# Autodesk Inventor assembly: hubRings
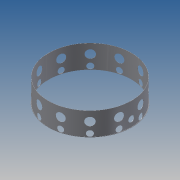
[picture p0: Inventor's stored thumbnail of the model, 180x180]
Saved by Autodesk Inventor 2014 SP1 (Build 180222100, 222)
## iProperties
Created: 2014-12-05
Part Number: hubRings
Document SubType Name: Assembly
Designer: Dave
Author: Dave
## Documents named in this file (4)
- C:\Users\Dave\Desktop\hera-cad\hub\hubRings.iam
- C:\Users\Dave\Desktop\hera-cad\hub\ringOuterPanel.ipt
- C:\Users\Dave\Desktop\hera-cad\hub\ringOuterPanel_MIR.ipt
- C:\Users\Dave\Desktop\hera-cad\hub\hubGuideRingOuter.ipt
## Components (3 placed, 3 different names)
1. ringOuterPanel:1 — Flush:1
2. ringOuterPanel_MIR:1 — Flush:1, Mate:1
3. hubGuideRingOuter:1 — Mate:1
## Relationships (2: Flush 1, Mate 1)
- Flush:1: ringOuterPanel:1 ↔ ringOuterPanel_MIR:1
- Mate:1 (-3.81 mm): ringOuterPanel_MIR:1 ↔ hubGuideRingOuter:1
